# Autodesk Inventor assembly: 040205 DR-19-H6
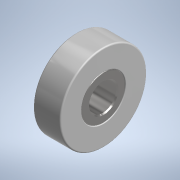
[picture p0: Inventor's stored thumbnail of the model, 180x180]
Saved by Autodesk Inventor 2022.3 (Build 263350000, 350)
## iProperties
Category: PARTsolutions
Company: TOKBEARING
Part Number: 040205 DR-19-H6
Catalog Web Link: www.cadenas.de
Description: DR-H-
Vendor: TOKBEARING
Document SubType Name: Assembly
Designer: partserver
Manufacturer: TOKBEARING
Mass: 3 g
Surface Area: 18.974 cm^2
Volume: 1.38361 cm^3
PSOL_IDENT_0: {$CADENAS_DATA\23d-libs\tok_bearing\d_series_bearings\dr_h_asmtab.prj},175 {VTYP=3D},{STYP=ASSTAB},{
PSOL_IDENT_1: NB=040205 DR-19-H6},{LINA=040205 DR-19-H6},{NN=DR-H},{DATE=16.12.2020 00:38:04},{GEOMDATE=19.02.2013
PSOL_IDENT_2: },{VERSION=},{LINEID=1520},{WBVAR=},{WBNUMERIC=}  {NB=040205 DR-19-H6},{LINA=040205 DR-19-H6},{KT=DU
PSOL_IDENT_3: MMY},{IDNR=},{CODE=040205},{PN=DR-19-H6},{D=19},{SD=6.0},{W=6.0},{W1=-},{W1X=0.000},{W2=-},{W2X=0.00
PSOL_IDENT_4: 0},{LOAD=49 (5)},{TYPE=10},{QTY=2.500},{GW=8.1},{BD=3.06},{OP=35.2622},{N=5},{R=5.615},{GP=3.12},{PP
PSOL_IDENT_5: ATH=dr_h/dr_h_asmtpl.prj}
NB: 040205 DR-19-H6
NN: DR-H
NBSYN: $CODE. $PN.
LINA: 040205 DR-19-H6
CATALOG: TOK, Inc
CODE: 040205
PN: DR-19-H6
D: 19
SD: 6
W: 6
W1: -
W2: -
LOAD: 49 (5)
TYPE: 10
QTY: 2.500
GW: 8.1
SUPPLIER: TOKBEARING
ARTICLENO: 040205 DR-19-H6
BOMINFO: 040205 DR-19-H6
CREATOR: CADENAS GmbH
Title: 040205 DR-19-H6
Author: Cadenas PARTsolutions
## Documents named in this file (5)
- C:\Users\YusukeKunita\Documents\GrabCAD\Development\BasicParts\Bearing\DR-19-H6\DR-19-H6.iam
- C:\Users\YusukeKunita\Documents\GrabCAD\Development\BasicParts\Bearing\DR-19-H6\DR-19-H6_ir.ipt
- C:\Users\YusukeKunita\Documents\GrabCAD\Development\BasicParts\Bearing\DR-19-H6\DR-19-H6_or.ipt
- C:\Users\YusukeKunita\Documents\GrabCAD\Development\BasicParts\Bearing\DR-19-H6\DR-19-H6_cage.ipt
- C:\Users\YusukeKunita\Documents\GrabCAD\Development\BasicParts\Bearing\DR-19-H6\DR-19-H6_ball.ipt
## Components (8 placed, 4 different names)
1. DR-19-H6_ir:1 — IR_OR_XY@1 <-> OR_IR_XY@2, IR_OR_Z@1 <-> OR_IR_Z@2
2. DR-19-H6_or:1 — IR_OR_XY@1 <-> OR_IR_XY@2, IR_OR_Z@1 <-> OR_IR_Z@2, OR_IR_XY@2 <-> Cage_OR_XY@3, OR_IR_Z@2 <-> Cage_OR_Z@3, OR_ball_1_XY@2 <-> Ball_OR_XY@4, OR_ball_1_Z@2 <-> Ball_OR_Z@4, OR_ball_1_YZ@2 <-> Ball_OR_YZ@4, OR_ball_2_XY@2 <-> Ball_OR_XY@5, OR_ball_2_Z@2 <-> Ball_OR_Z@5, OR_ball_2_YZ@2 <-> Ball_OR_YZ@5, OR_ball_3_XY@2 <-> Ball_OR_XY@6, OR_ball_3_Z@2 <-> Ball_OR_Z@6, OR_ball_3_YZ@2 <-> Ball_OR_YZ@6, OR_ball_4_XY@2 <-> Ball_OR_XY@7, OR_ball_4_Z@2 <-> Ball_OR_Z@7, OR_ball_4_YZ@2 <-> Ball_OR_YZ@7, OR_ball_5_XY@2 <-> Ball_OR_XY@8, OR_ball_5_Z@2 <-> Ball_OR_Z@8, OR_ball_5_YZ@2 <-> Ball_OR_YZ@8
3. DR-19-H6_cage:1 — OR_IR_XY@2 <-> Cage_OR_XY@3, OR_IR_Z@2 <-> Cage_OR_Z@3
4. DR-19-H6_ball:1 — OR_ball_1_XY@2 <-> Ball_OR_XY@4, OR_ball_1_Z@2 <-> Ball_OR_Z@4, OR_ball_1_YZ@2 <-> Ball_OR_YZ@4
5. DR-19-H6_ball:2 — OR_ball_2_XY@2 <-> Ball_OR_XY@5, OR_ball_2_Z@2 <-> Ball_OR_Z@5, OR_ball_2_YZ@2 <-> Ball_OR_YZ@5
6. DR-19-H6_ball:3 — OR_ball_3_XY@2 <-> Ball_OR_XY@6, OR_ball_3_Z@2 <-> Ball_OR_Z@6, OR_ball_3_YZ@2 <-> Ball_OR_YZ@6
7. DR-19-H6_ball:4 — OR_ball_4_XY@2 <-> Ball_OR_XY@7, OR_ball_4_Z@2 <-> Ball_OR_Z@7, OR_ball_4_YZ@2 <-> Ball_OR_YZ@7
8. DR-19-H6_ball:5 — OR_ball_5_XY@2 <-> Ball_OR_XY@8, OR_ball_5_Z@2 <-> Ball_OR_Z@8, OR_ball_5_YZ@2 <-> Ball_OR_YZ@8
## Relationships (19: Mate 12, Angle 5, Flush 2)
- IR_OR_XY@1 <-> OR_IR_XY@2 [Flush]: DR-19-H6_ir:1 ↔ DR-19-H6_or:1
- IR_OR_Z@1 <-> OR_IR_Z@2 [Mate]: DR-19-H6_ir:1 ↔ DR-19-H6_or:1
- OR_IR_XY@2 <-> Cage_OR_XY@3 [Flush]: DR-19-H6_or:1 ↔ DR-19-H6_cage:1
- OR_IR_Z@2 <-> Cage_OR_Z@3 [Mate]: DR-19-H6_or:1 ↔ DR-19-H6_cage:1
- OR_ball_1_XY@2 <-> Ball_OR_XY@4 [Mate]: DR-19-H6_or:1 ↔ DR-19-H6_ball:1
- OR_ball_1_Z@2 <-> Ball_OR_Z@4 [Mate]: DR-19-H6_or:1 ↔ DR-19-H6_ball:1
- OR_ball_1_YZ@2 <-> Ball_OR_YZ@4 [Angle] (0 deg): DR-19-H6_or:1 ↔ DR-19-H6_ball:1
- OR_ball_2_XY@2 <-> Ball_OR_XY@5 [Mate]: DR-19-H6_or:1 ↔ DR-19-H6_ball:2
- OR_ball_2_Z@2 <-> Ball_OR_Z@5 [Mate]: DR-19-H6_or:1 ↔ DR-19-H6_ball:2
- OR_ball_2_YZ@2 <-> Ball_OR_YZ@5 [Angle] (0 deg): DR-19-H6_or:1 ↔ DR-19-H6_ball:2
- OR_ball_3_XY@2 <-> Ball_OR_XY@6 [Mate]: DR-19-H6_or:1 ↔ DR-19-H6_ball:3
- OR_ball_3_Z@2 <-> Ball_OR_Z@6 [Mate]: DR-19-H6_or:1 ↔ DR-19-H6_ball:3
- OR_ball_3_YZ@2 <-> Ball_OR_YZ@6 [Angle] (0 deg): DR-19-H6_or:1 ↔ DR-19-H6_ball:3
- OR_ball_4_XY@2 <-> Ball_OR_XY@7 [Mate]: DR-19-H6_or:1 ↔ DR-19-H6_ball:4
- OR_ball_4_Z@2 <-> Ball_OR_Z@7 [Mate]: DR-19-H6_or:1 ↔ DR-19-H6_ball:4
- OR_ball_4_YZ@2 <-> Ball_OR_YZ@7 [Angle] (0 deg): DR-19-H6_or:1 ↔ DR-19-H6_ball:4
- OR_ball_5_XY@2 <-> Ball_OR_XY@8 [Mate]: DR-19-H6_or:1 ↔ DR-19-H6_ball:5
- OR_ball_5_Z@2 <-> Ball_OR_Z@8 [Mate]: DR-19-H6_or:1 ↔ DR-19-H6_ball:5
- OR_ball_5_YZ@2 <-> Ball_OR_YZ@8 [Angle] (0 deg): DR-19-H6_or:1 ↔ DR-19-H6_ball:5
